# Autodesk Inventor assembly: Leg_joint_slider_frame_SandBlastingJig_WearingImage
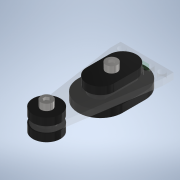
[picture p0: Inventor's stored thumbnail of the model, 180x180]
Saved by Autodesk Inventor 2022.3 (Build 263350000, 350)
## iProperties
Created: 2022-03-02
Part Number: Leg_joint_slider_frame_SandBlastingJig_WearingImage
Document SubType Name: Assembly
Designer: Masato Kubotera
Author: Masato Kubotera
## Documents named in this file (7)
- C:\Users\Masato\Desktop\SUSTAINA-OP\OptionParts\SandBlastingJig\Leg_joint_slider_frame_SandBlastingJig_WearingImage.iam
- C:\Users\Masato\Desktop\SUSTAINA-OP\LowerBody\Leg_joint\Leg_joint_slider_frame.ipt
- C:\Users\Masato\Desktop\SUSTAINA-OP\OptionParts\SandBlastingJig\Leg_joint_slider_frame_SandBlastingJig_axis_back.ipt
- C:\Users\Masato\Desktop\SUSTAINA-OP\OptionParts\SandBlastingJig\Leg_joint_slider_frame_SandBlastingJig_axis_front.ipt
- C:\Users\Masato\Desktop\SUSTAINA-OP\OptionParts\SandBlastingJig\Leg_joint_slider_frame_SandBlastingJig_slider_back.ipt
- C:\Users\Masato\Desktop\SUSTAINA-OP\OptionParts\SandBlastingJig\Leg_joint_slider_frame_SandBlastingJig_slider_front.ipt
- C:\Users\Masato\Desktop\SUSTAINA-OP\ReadyMade\Screw\M3-10.ipt
## Components (7 placed, 6 different names)
1. Leg_joint_slider_frame:1 — 挿入:1, 挿入:2, 挿入:3, 挿入:4, 挿入:5, 挿入:6, メイト:1, メイト:2, フラッシュ:1
2. Leg_joint_slider_frame_SandBlastingJig_axis_back:1 — 挿入:4, 挿入:7
3. Leg_joint_slider_frame_SandBlastingJig_axis_front:1 — 挿入:3
4. Leg_joint_slider_frame_SandBlastingJig_slider_back:1 — 挿入:5, 挿入:6, 挿入:8
5. Leg_joint_slider_frame_SandBlastingJig_slider_front:1 — 挿入:1, 挿入:2
6. M3-10:1 — 挿入:7
7. M3-10:2 — 挿入:8
## Relationships (11: Insert 8, Mate 2, Flush 1)
- 挿入:1 [Insert]: Leg_joint_slider_frame:1 ↔ Leg_joint_slider_frame_SandBlastingJig_slider_front:1
- 挿入:2 [Insert]: Leg_joint_slider_frame:1 ↔ Leg_joint_slider_frame_SandBlastingJig_slider_front:1
- 挿入:3 [Insert]: Leg_joint_slider_frame:1 ↔ Leg_joint_slider_frame_SandBlastingJig_axis_front:1
- 挿入:4 [Insert]: Leg_joint_slider_frame:1 ↔ Leg_joint_slider_frame_SandBlastingJig_axis_back:1
- 挿入:5 [Insert]: Leg_joint_slider_frame:1 ↔ Leg_joint_slider_frame_SandBlastingJig_slider_back:1
- 挿入:6 [Insert]: Leg_joint_slider_frame:1 ↔ Leg_joint_slider_frame_SandBlastingJig_slider_back:1
- 挿入:7 [Insert]: Leg_joint_slider_frame_SandBlastingJig_axis_back:1 ↔ M3-10:1
- 挿入:8 [Insert]: Leg_joint_slider_frame_SandBlastingJig_slider_back:1 ↔ M3-10:2
- メイト:1 [Mate]: Leg_joint_slider_frame:1
- メイト:2 [Mate]: Leg_joint_slider_frame:1
- フラッシュ:1 [Flush]: Leg_joint_slider_frame:1
